# Autodesk Inventor assembly: New_battery
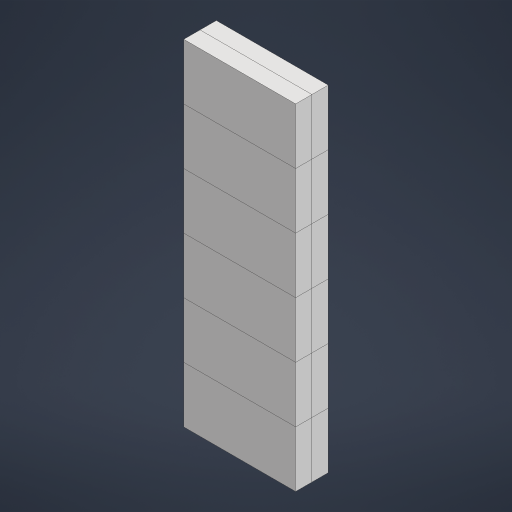
[picture p0: Inventor's stored thumbnail of the model, 512x512]
Saved by Autodesk Inventor 2024 (Build 280153000, 153)
## iProperties
Created: 2024-02-29
Part Number: New_battery
Document SubType Name: Assembly
Designer: calvi
Author: calvi
## Documents named in this file (2)
- C:\Users\calvi\OneDrive\Robocup Rescue\Chassis\Electronics Box\EBox-Parts\New_battery - Copy.iam
- C:\Users\calvi\OneDrive\Robocup Rescue\Chassis\Electronics Box\EBox-Parts\Battery_Cell.ipt
## Components (12 placed, 1 different names)
1. Battery_Cell:1 — Mate:8, Flush:15, Flush:17, Mate:19, Flush:31, Flush:34
2. Battery_Cell:2 — Mate:7, Flush:12, Flush:13, Mate:14, Flush:24, Flush:25
3. Battery_Cell:3 — Mate:7, Flush:12, Flush:13
4. Battery_Cell:4 — Mate:9, Flush:18, Flush:32, Flush:34
5. Battery_Cell:5 — Mate:8, Flush:15, Flush:17, Flush:30, Mate:20, Flush:33
6. Battery_Cell:6 — Mate:10, Flush:20, Flush:21
7. Battery_Cell:7 — Mate:3, Flush:6, Flush:7, Mate:11, Mate:13, Flush:22, Flush:23, Flush:28, Flush:29
8. Battery_Cell:8 — Mate:3, Flush:6, Flush:7, Mate:17
9. Battery_Cell:9 — Mate:10, Flush:20, Flush:21, Mate:11, Mate:13, Flush:22, Flush:23, Mate:14, Flush:24, Flush:25
10. Battery_Cell:10 — Mate:9, Flush:18, Flush:32, Mate:20, Flush:33
11. Battery_Cell:11 — Mate:17, Mate:18, Flush:26, Flush:27, Mate:19, Flush:30
12. Battery_Cell:12 — Mate:18, Flush:26, Flush:27, Flush:28, Flush:29, Flush:31
## Relationships (34: Flush 22, Mate 12)
- Mate:3: Battery_Cell:7 ↔ Battery_Cell:8
- Flush:6: Battery_Cell:7 ↔ Battery_Cell:8
- Flush:7: Battery_Cell:7 ↔ Battery_Cell:8
- Mate:7: Battery_Cell:2 ↔ Battery_Cell:3
- Flush:12: Battery_Cell:2 ↔ Battery_Cell:3
- Flush:13: Battery_Cell:2 ↔ Battery_Cell:3
- Mate:8: Battery_Cell:1 ↔ Battery_Cell:5
- Flush:15: Battery_Cell:1 ↔ Battery_Cell:5
- Flush:17: Battery_Cell:1 ↔ Battery_Cell:5
- Mate:9: Battery_Cell:4 ↔ Battery_Cell:10
- Flush:18: Battery_Cell:4 ↔ Battery_Cell:10
- Mate:10: Battery_Cell:6 ↔ Battery_Cell:9
- Flush:20: Battery_Cell:6 ↔ Battery_Cell:9
- Flush:21: Battery_Cell:6 ↔ Battery_Cell:9
- Mate:11: Battery_Cell:7 ↔ Battery_Cell:9
- Mate:13: Battery_Cell:7 ↔ Battery_Cell:9
- Flush:22: Battery_Cell:7 ↔ Battery_Cell:9
- Flush:23: Battery_Cell:7 ↔ Battery_Cell:9
- Mate:14: Battery_Cell:2 ↔ Battery_Cell:9
- Flush:24: Battery_Cell:2 ↔ Battery_Cell:9
- Flush:25: Battery_Cell:2 ↔ Battery_Cell:9
- Mate:17: Battery_Cell:8 ↔ Battery_Cell:11
- Mate:18: Battery_Cell:11 ↔ Battery_Cell:12
- Flush:26: Battery_Cell:11 ↔ Battery_Cell:12
- Flush:27: Battery_Cell:11 ↔ Battery_Cell:12
- Flush:28: Battery_Cell:7 ↔ Battery_Cell:12
- Flush:29: Battery_Cell:7 ↔ Battery_Cell:12
- Mate:19: Battery_Cell:1 ↔ Battery_Cell:11
- Flush:30: Battery_Cell:5 ↔ Battery_Cell:11
- Flush:31: Battery_Cell:1 ↔ Battery_Cell:12
- Flush:32: Battery_Cell:4 ↔ Battery_Cell:10
- Mate:20: Battery_Cell:5 ↔ Battery_Cell:10
- Flush:33: Battery_Cell:5 ↔ Battery_Cell:10
- Flush:34: Battery_Cell:1 ↔ Battery_Cell:4
